# Autodesk Inventor assembly: ruka
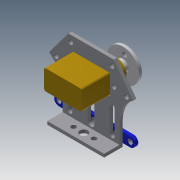
[picture p0: Inventor's stored thumbnail of the model, 180x180]
Saved by Autodesk Inventor 2013 (Build 170138000, 138)
## iProperties
Created: 2013-03-08
Part Number: ruka
Document SubType Name: Assembly
Designer: idle-rug
Author: idle-rug
## Documents named in this file (5)
- C:\Users\Petr\Documents\Inventor\robotic arm\ruka.iam
- C:\Users\Petr\Documents\Inventor\robotic arm\tahlo4(2).ipt
- C:\Users\Petr\Documents\Inventor\robotic arm\ruka_zak, deska2.ipt
- C:\Users\Petr\Documents\Inventor\robotic arm\micro_servo.ipt
- C:\Users\Petr\Documents\Inventor\robotic arm\paka2_micro.ipt
## Components (4 placed, 4 different names)
1. tahlo4(2):2 — Mate:5
2. ruka_zak, deska2:1 — Mate:2, Mate:3, Mate:5, Mate:6
3. micro_servo:1 — Mate:2, Mate:3, Mate:6, Mate:7, Mate:8
4. paka2_micro:1 — Mate:7, Mate:8
## Relationships (6: Mate 6)
- Mate:2: ruka_zak, deska2:1 ↔ micro_servo:1
- Mate:3: ruka_zak, deska2:1 ↔ micro_servo:1
- Mate:5: tahlo4(2):2 ↔ ruka_zak, deska2:1
- Mate:6: ruka_zak, deska2:1 ↔ micro_servo:1
- Mate:7: micro_servo:1 ↔ paka2_micro:1
- Mate:8: micro_servo:1 ↔ paka2_micro:1
